# Autodesk Inventor assembly: Spreader assy
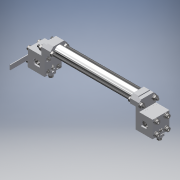
[picture p0: Inventor's stored thumbnail of the model, 180x180]
Saved by Autodesk Inventor 2018 (Build 220112000, 112)
## iProperties
Created: 2017-10-02
Part Number: Spreader assy
Document SubType Name: Assembly
Designer: Gabriel Smolnycki
Author: Gabriel Smolnycki
## Documents named in this file (14)
- E:\planb\mechanics\Subassemblies\Spreader assy.iam
- E:\planb\mechanics\Spreader\Spreader Frame.ipt
- E:\planb\mechanics\Spreader\Spreader Linear Bearing Clamp.ipt
- E:\planb\mechanics\Hardware\8x25 Linear Bearing (63255K45).ipt
- E:\planb\mechanics\Hardware\M4 SS Locknut.ipt
- E:\planb\mechanics\Hardware\M4 SS Washer.ipt
- E:\planb\mechanics\Hardware\M4 SS Nut.ipt
- E:\planb\mechanics\Hardware\M4x16 SS SHCS.ipt
- E:\planb\mechanics\Spreader\Spreader Belt Clamp.ipt
- E:\planb\mechanics\Spreader\Spreader.ipt
- E:\planb\mechanics\Spreader\Spreader Holder.ipt
- E:\planb\mechanics\Spreader\Spreader Flag.ipt
- E:\planb\mechanics\Hardware\M4x35 SS SHCS.ipt
- E:\planb\mechanics\Spreader\Spreader Threaded Rod M4.ipt
## Components (62 placed, 13 different names)
1. Spreader Frame:1 — Insert:2, Insert:3, Insert:4, Mate:1, Insert:5, Mate:2, Insert:6, Mate:3, Insert:7, Mate:4, Tangent:1, Mate:6, Mate:7, Insert:45, Insert:46, Insert:58, Insert:59
2. Spreader Linear Bearing Clamp:1 — Insert:1, Insert:2, Insert:3, Insert:8, Insert:9, Insert:10, Insert:11, Insert:16, Mate:5, Insert:19
3. 8x25 Linear Bearing (63255K45):1 — Insert:1
4. M4 SS Locknut:1 — Insert:6, Mate:3
5. M4 SS Locknut:2 — Insert:7, Mate:4
6. M4 SS Locknut:3 — Insert:4, Mate:1
7. M4 SS Locknut:4 — Insert:5, Mate:2
8. M4 SS Washer:1 — Insert:8
9. M4 SS Washer:2 — Insert:9
10. M4 SS Washer:3 — Insert:10
11. M4 SS Washer:4 — Insert:11
12. M4x35 SS SHCS:1
13. M4x35 SS SHCS:2
14. M4x35 SS SHCS:3
15. M4x35 SS SHCS:4
16. M4 SS Nut:1 — Mate:6, Mate:7, Insert:22
17. M4 SS Nut:2 — Mate:5, Insert:19
18. M4 SS Washer:5 — Insert:18, Insert:20
19. M4 SS Washer:6 — Insert:17, Insert:21
20. M4x16 SS SHCS:1 — Insert:21
21. M4x16 SS SHCS:2 — Insert:20, Insert:22
22. Spreader Belt Clamp:1 — Insert:16, Tangent:1, Insert:17, Insert:18
23. Spreader Frame:2 — Insert:48, Insert:49, Insert:60, Insert:61
24. Spreader Linear Bearing Clamp:2 — Insert:52, Flush:1
25. 8x25 Linear Bearing (63255K45):2
26. M4 SS Locknut:5
27. M4 SS Locknut:6
28. M4 SS Locknut:7
29. M4 SS Locknut:8
30. M4 SS Washer:7
31. M4 SS Washer:8
32. M4 SS Washer:9 — Insert:53
33. M4 SS Washer:10
34. M4x35 SS SHCS:5
35. M4x35 SS SHCS:6
36. M4x35 SS SHCS:7
37. M4x35 SS SHCS:8
38. M4 SS Nut:3
39. M4 SS Nut:4
40. M4 SS Washer:11
41. M4 SS Washer:12
42. M4x16 SS SHCS:3
43. M4x16 SS SHCS:4
44. Spreader Belt Clamp:2
45. Spreader:1 — Insert:47, Insert:50
46. Spreader Holder:1 — Insert:48, Insert:49, Insert:50, Insert:51, Insert:70, Insert:71
47. Spreader Holder:2 — Insert:45, Insert:46, Insert:47, Insert:51, Insert:72, Insert:73
48. Spreader Flag:1 — Insert:52, Insert:53, Flush:1
49. M4 SS Washer:15 — Insert:58, Insert:69
50. M4 SS Washer:16 — Insert:59, Insert:68
51. M4 SS Washer:17 — Insert:61, Insert:63
52. M4 SS Washer:18 — Insert:60, Insert:62
53. M4 SS Nut:5 — Insert:62, Insert:74
54. M4 SS Nut:6 — Insert:63, Insert:75
55. M4 SS Nut:7 — Insert:71
56. M4 SS Nut:8 — Insert:70
57. M4 SS Nut:9 — Insert:68
58. M4 SS Nut:10 — Insert:69
59. M4 SS Nut:11 — Insert:73
60. M4 SS Nut:12 — Insert:72
61. Spreader Threaded Rod M4:1 — Insert:75
62. Spreader Threaded Rod M4:2 — Insert:74
## Relationships (83: Insert 66, Mate 14, Tangent 2, Flush 1)
- Insert:1 (0.25 mm): Spreader Linear Bearing Clamp:1 ↔ 8x25 Linear Bearing (63255K45):1
- Insert:2: Spreader Frame:1 ↔ Spreader Linear Bearing Clamp:1
- Insert:3: Spreader Frame:1 ↔ Spreader Linear Bearing Clamp:1
- Insert:4: Spreader Frame:1 ↔ M4 SS Locknut:3
- Mate:1: Spreader Frame:1 ↔ M4 SS Locknut:3
- Insert:5: Spreader Frame:1 ↔ M4 SS Locknut:4
- Mate:2: Spreader Frame:1 ↔ M4 SS Locknut:4
- Insert:6: Spreader Frame:1 ↔ M4 SS Locknut:1
- Mate:3: Spreader Frame:1 ↔ M4 SS Locknut:1
- Insert:7: Spreader Frame:1 ↔ M4 SS Locknut:2
- Mate:4: Spreader Frame:1 ↔ M4 SS Locknut:2
- Insert:8: Spreader Linear Bearing Clamp:1 ↔ M4 SS Washer:1
- Insert:9: Spreader Linear Bearing Clamp:1 ↔ M4 SS Washer:2
- Insert:10: Spreader Linear Bearing Clamp:1 ↔ M4 SS Washer:3
- Insert:11: Spreader Linear Bearing Clamp:1 ↔ M4 SS Washer:4
- [Insert]: M4 SS Washer:2 ↔ M4x35 SS SHCS:2
- [Insert]: M4 SS Washer:1 ↔ M4x35 SS SHCS:4
- [Insert]: M4 SS Washer:3 ↔ M4x35 SS SHCS:1
- [Insert]: M4 SS Washer:4 ↔ M4x35 SS SHCS:3
- Insert:16: Spreader Linear Bearing Clamp:1 ↔ Spreader Belt Clamp:1
- Tangent:1: Spreader Frame:1 ↔ Spreader Belt Clamp:1
- Insert:17: M4 SS Washer:6 ↔ Spreader Belt Clamp:1
- Insert:18: M4 SS Washer:5 ↔ Spreader Belt Clamp:1
- Mate:5: Spreader Linear Bearing Clamp:1 ↔ M4 SS Nut:2
- Insert:19: Spreader Linear Bearing Clamp:1 ↔ M4 SS Nut:2
- Insert:20: M4 SS Washer:5 ↔ M4x16 SS SHCS:2
- Insert:21: M4 SS Washer:6 ↔ M4x16 SS SHCS:1
- Mate:6: Spreader Frame:1 ↔ M4 SS Nut:1
- Mate:7: Spreader Frame:1 ↔ M4 SS Nut:1
- Insert:22: M4 SS Nut:1 ↔ M4x16 SS SHCS:2
- [Insert] (0.25 mm): Spreader Linear Bearing Clamp:2 ↔ 8x25 Linear Bearing (63255K45):2
- [Insert]: Spreader Frame:2 ↔ Spreader Linear Bearing Clamp:2
- [Insert]: Spreader Frame:2 ↔ Spreader Linear Bearing Clamp:2
- [Insert]: Spreader Frame:2 ↔ M4 SS Locknut:7
- [Mate]: Spreader Frame:2 ↔ M4 SS Locknut:7
- [Insert]: Spreader Frame:2 ↔ M4 SS Locknut:8
- [Mate]: Spreader Frame:2 ↔ M4 SS Locknut:8
- [Insert]: Spreader Frame:2 ↔ M4 SS Locknut:5
- [Mate]: Spreader Frame:2 ↔ M4 SS Locknut:5
- [Insert]: Spreader Frame:2 ↔ M4 SS Locknut:6
- [Mate]: Spreader Frame:2 ↔ M4 SS Locknut:6
- [Insert]: Spreader Linear Bearing Clamp:2 ↔ M4 SS Washer:7
- [Insert]: Spreader Linear Bearing Clamp:2 ↔ M4 SS Washer:8
- [Insert]: Spreader Linear Bearing Clamp:2 ↔ M4 SS Washer:10
- [Insert]: M4 SS Washer:8 ↔ M4x35 SS SHCS:6
- [Insert]: M4 SS Washer:7 ↔ M4x35 SS SHCS:8
- [Insert]: M4 SS Washer:9 ↔ M4x35 SS SHCS:5
- [Insert]: M4 SS Washer:10 ↔ M4x35 SS SHCS:7
- [Insert]: Spreader Linear Bearing Clamp:2 ↔ Spreader Belt Clamp:2
- [Tangent]: Spreader Frame:2 ↔ Spreader Belt Clamp:2
- [Insert]: M4 SS Washer:12 ↔ Spreader Belt Clamp:2
- [Insert]: M4 SS Washer:11 ↔ Spreader Belt Clamp:2
- [Mate]: Spreader Linear Bearing Clamp:2 ↔ M4 SS Nut:4
- [Insert]: Spreader Linear Bearing Clamp:2 ↔ M4 SS Nut:4
- [Insert]: M4 SS Washer:11 ↔ M4x16 SS SHCS:4
- [Insert]: M4 SS Washer:12 ↔ M4x16 SS SHCS:3
- [Mate]: Spreader Frame:2 ↔ M4 SS Nut:3
- [Mate]: Spreader Frame:2 ↔ M4 SS Nut:3
- [Insert]: M4 SS Nut:3 ↔ M4x16 SS SHCS:4
- Insert:45: Spreader Frame:1 ↔ Spreader Holder:2
- Insert:46: Spreader Frame:1 ↔ Spreader Holder:2
- Insert:47 (0.8 mm): Spreader:1 ↔ Spreader Holder:2
- Insert:48: Spreader Frame:2 ↔ Spreader Holder:1
- Insert:49: Spreader Frame:2 ↔ Spreader Holder:1
- Insert:50 (0.8 mm): Spreader:1 ↔ Spreader Holder:1
- Insert:51: Spreader Holder:1 ↔ Spreader Holder:2
- Insert:52: Spreader Linear Bearing Clamp:2 ↔ Spreader Flag:1
- Insert:53: M4 SS Washer:9 ↔ Spreader Flag:1
- Flush:1: Spreader Linear Bearing Clamp:2 ↔ Spreader Flag:1
- Insert:58: Spreader Frame:1 ↔ M4 SS Washer:15
- Insert:59: Spreader Frame:1 ↔ M4 SS Washer:16
- Insert:60: Spreader Frame:2 ↔ M4 SS Washer:18
- Insert:61: Spreader Frame:2 ↔ M4 SS Washer:17
- Insert:62: M4 SS Washer:18 ↔ M4 SS Nut:5
- Insert:63: M4 SS Washer:17 ↔ M4 SS Nut:6
- Insert:68: M4 SS Washer:16 ↔ M4 SS Nut:9
- Insert:69: M4 SS Washer:15 ↔ M4 SS Nut:10
- Insert:70: Spreader Holder:1 ↔ M4 SS Nut:8
- Insert:71: Spreader Holder:1 ↔ M4 SS Nut:7
- Insert:72: Spreader Holder:2 ↔ M4 SS Nut:12
- Insert:73: Spreader Holder:2 ↔ M4 SS Nut:11
- Insert:74 (-4.7 mm): M4 SS Nut:5 ↔ Spreader Threaded Rod M4:2
- Insert:75 (-4.7 mm): M4 SS Nut:6 ↔ Spreader Threaded Rod M4:1
## Named parameters: d32_d24 = 0 mm, d33_d25 = 0 mm, d34_d26 = 0 mm, d35_d27 = 0 mm, d36_d28 = 0 mm, d37_d29 = 0 mm, d38_d30 = 0 mm, d39_d31 = 0 mm, d40_d17 = 0 mm, d41_d18 = 0 mm, d42_d19 = 0 mm, d43_d20 = 0 mm, d44_d21 = 0 mm, d45_d22 = 0 mm, d46_d23 = 0 mm, d47_d2 = 0 mm, d48_d3 = 0 mm, d49_d4 = 0 mm, d50_d5 = 0 mm, d51_d6 = 0 mm, d52_d7 = 0 mm, d53_d8 = 0 mm, d54_d0 = 0.25 mm, d55_d1 = 0 mm, d56_d9 = 0 mm, d57_d10 = 0 mm, d58_d11 = 0 mm, d59_d12 = 0 mm, d61_d14 = 0 mm, d62_d15 = 0 mm, d63_d16 = 0 mm
